# Autodesk Inventor assembly: Second Stage
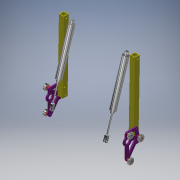
[picture p0: Inventor's stored thumbnail of the model, 180x180]
Saved by Autodesk Inventor 2017 SP1 (Build 210196100, 196)
## iProperties
Created: 2018-01-18
Part Number: Second Stage
Document SubType Name: Assembly
Designer: Ben
Mass: 9979.66 g
Surface Area: 70095.8 cm^2
Volume: 103427 cm^3
Density: 0.0964899 g/cm^3
Author: Ben
## Documents named in this file (5)
- C:\Users\Ben\Desktop\Projects\2018 Robot\Cube Lift\Second Stage.iam
- C:\Users\Ben\Desktop\Projects\2018 Robot\Cube Lift\roller bushing.iam
- C:\Users\Ben\Desktop\Projects\2018 Robot\Cube Lift\carriage plate for intake.ipt
- C:\Users\Ben\Desktop\Projects\2018 Robot\Cube Lift\cylinder arm.ipt
- C:\Users\Ben\Desktop\Projects\2018 Robot\Cube Lift\Cylinder.iam
## Components (12 placed, 4 different names)
1. roller bushing:4 [sub-assembly] — Insert:11
2. roller bushing:5 [sub-assembly] — Mate:53
3. roller bushing:6 [sub-assembly] — Mate:56
4. carriage plate for intake:1 — Mate:53, Insert:11, Mate:56, Insert:12, Insert:16
5. cylinder arm:1 — Insert:12, Insert:16, Insert:29
6. carriage plate for intake:2 — Insert:22, Insert:23, Insert:24, Insert:27, Insert:28
7. roller bushing:9 [sub-assembly] — Insert:24
8. roller bushing:11 [sub-assembly] — Insert:22
9. roller bushing:12 [sub-assembly] — Insert:23
10. cylinder arm:2 — Insert:27, Insert:28, Insert:30
11. Cylinder:1 [sub-assembly] — Insert:29, Angle:1
12. Cylinder:2 [sub-assembly] — Insert:30, Angle:1
## Relationships (13: Insert 10, Mate 2, Angle 1)
- Mate:53: roller bushing:5 ↔ carriage plate for intake:1
- Insert:11: roller bushing:4 ↔ carriage plate for intake:1
- Mate:56: roller bushing:6 ↔ carriage plate for intake:1
- Insert:12: carriage plate for intake:1 ↔ cylinder arm:1
- Insert:16: carriage plate for intake:1 ↔ cylinder arm:1
- Insert:22: carriage plate for intake:2 ↔ roller bushing:11
- Insert:23: carriage plate for intake:2 ↔ roller bushing:12
- Insert:24: carriage plate for intake:2 ↔ roller bushing:9
- Insert:27: carriage plate for intake:2 ↔ cylinder arm:2
- Insert:28: carriage plate for intake:2 ↔ cylinder arm:2
- Insert:29 (25.4 mm): cylinder arm:1 ↔ Cylinder:1
- Insert:30 (25.4 mm): cylinder arm:2 ↔ Cylinder:2
- Angle:1 (0 deg): Cylinder:1 ↔ Cylinder:2
